# Autodesk Inventor assembly: Ball Launcher Mechanism
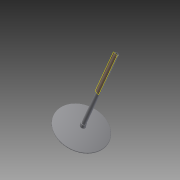
[picture p0: Inventor's stored thumbnail of the model, 180x180]
Saved by Autodesk Inventor 2014 SP1 (Build 180222100, 222)
## iProperties
Created: 2014-01-06
Part Number: Ball Launcher Mechanism
Document SubType Name: Assembly
Designer: Andrew Toennies
Mass: 115.496 g
Surface Area: 574.912 cm^2
Volume: 115.496 cm^3
Density: 1 g/cm^3
Author: Andrew Toennies
## Documents named in this file (3)
- C:\Users\Arpan\Documents\GitHub\2014buildCAD\Shooter\Ball Launcher Mechanism.iam
- C:\Users\Arpan\Documents\GitHub\2014buildCAD\Shooter\Launcher.ipt
- C:\Users\Arpan\Documents\GitHub\2014buildCAD\Shooter\Launcher Crossbow.ipt
## Components (2 placed, 2 different names)
1. Launcher:1 — Mate:1, Mate:2
2. Launcher Crossbow:1 — Mate:1, Mate:2
## Relationships (2: Mate 2)
- Mate:1: Launcher:1 ↔ Launcher Crossbow:1
- Mate:2: Launcher:1 ↔ Launcher Crossbow:1
